# Autodesk Inventor assembly: Chassis-ver1-1111-2021
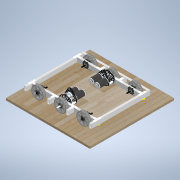
[picture p0: Inventor's stored thumbnail of the model, 180x180]
Saved by Autodesk Inventor 2020 (Build 240168000, 168)
## iProperties
Created: 2021-01-26
Part Number: Chassis-ver1-1111-2021
Document SubType Name: Assembly
Designer: Caitlin
Author: Caitlin
## Documents named in this file (14)
- D:\PHRC CADD 2021\PHRC CADD\2020 Infinite Recharge\2021 Infinite Recharge\Chassis\Chassis-ver1-1111-2021.iam
- D:\PHRC CADD 2021\PHRC CADD\2020 Infinite Recharge\Platform.ver1-1111-2020.ipt
- D:\PHRC CADD 2021\PHRC CADD\2020 Infinite Recharge\Chassis\Parts\2x1 20in Alluminum.ver1-1111-2019.ipt
- D:\PHRC CADD 2021\PHRC CADD\2020 Infinite Recharge\Chassis\Parts\2x1 20in Alluminum with Cal Drop.ver1-1111-2019.ipt
- D:\PHRC CADD 2021\PHRC CADD\Resources\VEXpro Resources\Gussets\ChassisGusset-1111-2016.ipt
- D:\PHRC CADD 2021\PHRC CADD\2020 Infinite Recharge\Chassis\Parts\2x1 2in Alluminum Block.ver1-1111-2019.ipt
- D:\PHRC CADD 2021\PHRC CADD\Resources\VEXpro Resources\Bearings\0.5inHexFlangedBearing(1.125inx0.313in)-1111-2016.ipt
- D:\PHRC CADD 2021\PHRC CADD\Resources\VEXpro Resources\Spacers\0.5inAcetalSpace(0.5inHex)-1111-2016.ipt
- D:\PHRC CADD 2021\PHRC CADD\Resources\VEXpro Resources\Versa Motion\VersaBlockKit-1111-2016.ipt
- D:\PHRC CADD 2021\PHRC CADD\Resources\VEXpro Resources\Gearboxes\WCP SS Gearbox\SS-Gearbox.iam
- D:\PHRC CADD 2021\PHRC CADD\Resources\VEXpro Resources\Shafts\0.5inThunderHexShaft(8)-1111-2016.ipt
- D:\PHRC CADD 2021\PHRC CADD\Resources\VEXpro Resources\Wheels\6 inch\6x1inTractionWheel-1111-2016.iam
- D:\PHRC CADD 2021\PHRC CADD\2020 Infinite Recharge\Chassis\Parts\BumperMount1-ver1-1111-2019.ipt
- D:\PHRC CADD 2021\PHRC CADD\2020 Infinite Recharge\Chassis\Parts\ElectricalBoard.ver2-1111-2020.ipt
## Components (51 placed, 13 different names)
1. Platform.ver1-1111-2020:1 — Mate:1, Flush:1, Flush:2
2. 2x1 20in Alluminum.ver1-1111-2019:1 — Mate:1, Flush:1, Flush:2, Mate:2, Mate:3, Flush:3, Mate:4, Mate:5, Flush:4, Mate:8, Flush:6, Mate:9, Flush:8, Mate:14, Mate:40, Flush:23, Mate:41, Flush:27, Mate:46
3. 2x1 20in Alluminum with Cal Drop.ver1-1111-2019:1 — Mate:2, Mate:3, Flush:3, Mate:6, Mate:7, Flush:5, Flush:7, Flush:11, Mate:12, Mate:13, Mate:15, Mate:16, Flush:14, Mate:19, Flush:16, Cylindrical:3, Mate:30, Cylindrical:4, Mate:31, Cylindrical:7, Mate:34, Cylindrical:8, Mate:35, Angle:5, Angle:6, Angle:7, Angle:8, Cylindrical:9, Mate:36, Angle:13, Flush:25, Flush:26, Mate:43, Mate:44, Mate:45, Flush:28
4. 2x1 20in Alluminum with Cal Drop.ver1-1111-2019:2 — Mate:4, Mate:5, Flush:4, Flush:9, Flush:13, Mate:20, Mate:21, Mate:23, Mate:24, Mate:26, Flush:18, Mate:27, Flush:20, Cylindrical:1, Mate:28, Cylindrical:2, Mate:29, Cylindrical:5, Mate:32, Cylindrical:6, Mate:33, Angle:9, Angle:10, Angle:11, Angle:12, Cylindrical:10, Mate:37, Angle:14, Mate:38, Flush:22, Mate:39, Flush:24, Mate:42
5. 2x1 20in Alluminum.ver1-1111-2019:2 — Mate:6, Mate:7, Flush:5, Mate:10, Flush:10, Mate:11, Flush:12, Mate:22
6. ChassisGusset-1111-2016:1 — Mate:8, Flush:6, Flush:7
7. ChassisGusset-1111-2016:2 — Mate:9, Flush:8, Flush:9
8. ChassisGusset-1111-2016:3 — Mate:10, Flush:10, Flush:11
9. ChassisGusset-1111-2016:4 — Mate:11, Flush:12, Flush:13
10. 2x1 2in Alluminum Block.ver1-1111-2019:1 — Mate:12, Mate:13, Mate:14, Mate:17, Flush:17
11. 2x1 2in Alluminum Block.ver1-1111-2019:2 — Mate:15, Mate:16, Mate:17, Mate:18, Flush:15
12. ChassisGusset-1111-2016:5 — Mate:18, Flush:14, Flush:15
13. ChassisGusset-1111-2016:6 — Mate:19, Flush:16, Flush:17
14. 2x1 2in Alluminum Block.ver1-1111-2019:3 — Mate:20, Mate:21, Mate:22, Mate:25, Flush:19
15. 2x1 2in Alluminum Block.ver1-1111-2019:4 — Mate:23, Mate:24, Mate:25, Flush:21
16. ChassisGusset-1111-2016:7 — Mate:26, Flush:18, Flush:19
17. ChassisGusset-1111-2016:8 — Mate:27, Flush:20, Flush:21
18. 0.5inHexFlangedBearing(1.125inx0.313in)-1111-2016:1 — Cylindrical:1, Mate:28, Rotational:11
19. 0.5inHexFlangedBearing(1.125inx0.313in)-1111-2016:2 — Cylindrical:2, Mate:29, Rotational:12
20. 0.5inHexFlangedBearing(1.125inx0.313in)-1111-2016:3 — Cylindrical:3, Mate:30, Rotational:8
21. 0.5inHexFlangedBearing(1.125inx0.313in)-1111-2016:4 — Cylindrical:4, Mate:31, Rotational:7
22. 0.5inHexFlangedBearing(1.125inx0.313in)-1111-2016:5 — Cylindrical:5, Mate:32, Rotational:3, Angle:3, Rotational:9
23. 0.5inHexFlangedBearing(1.125inx0.313in)-1111-2016:6 — Cylindrical:6, Mate:33, Rotational:4, Angle:4, Rotational:10, Cylindrical:14
24. 0.5inHexFlangedBearing(1.125inx0.313in)-1111-2016:7 — Cylindrical:7, Mate:34, Rotational:1, Angle:1, Rotational:5
25. 0.5inHexFlangedBearing(1.125inx0.313in)-1111-2016:8 — Cylindrical:8, Mate:35, Rotational:2, Angle:2, Rotational:6
26. 0.5inAcetalSpace(0.5inHex)-1111-2016:1 — Rotational:1, Angle:1, Cylindrical:17
27. 0.5inAcetalSpace(0.5inHex)-1111-2016:2 — Rotational:2, Angle:2, Cylindrical:16
28. 0.5inAcetalSpace(0.5inHex)-1111-2016:3 — Rotational:3, Angle:3, Cylindrical:12
29. 0.5inAcetalSpace(0.5inHex)-1111-2016:4 — Rotational:4, Angle:4
30. VersaBlockKit-1111-2016:1 — Rotational:5, Angle:5
31. VersaBlockKit-1111-2016:2 — Rotational:6, Angle:6
32. VersaBlockKit-1111-2016:3 — Rotational:7, Angle:7
33. VersaBlockKit-1111-2016:4 — Rotational:8, Angle:8
34. VersaBlockKit-1111-2016:5 — Rotational:9, Angle:9
35. VersaBlockKit-1111-2016:6 — Rotational:10, Angle:10
36. VersaBlockKit-1111-2016:7 — Rotational:11, Angle:11
37. VersaBlockKit-1111-2016:8 — Rotational:12, Angle:12
38. SS-Gearbox:1 [sub-assembly] — Cylindrical:9, Mate:36, Angle:13, Cylindrical:20
39. SS-Gearbox:2 [sub-assembly] — Cylindrical:10, Mate:37, Angle:14, Cylindrical:11
40. 0.5inThunderHexShaft(8)-1111-2016:1 — Cylindrical:12, Flush:22, Cylindrical:13, Angle:15
41. 6x1inTractionWheel-1111-2016:1 [sub-assembly] — Cylindrical:11, Mate:38
42. 6x1inTractionWheel-1111-2016:2 [sub-assembly] — Cylindrical:13, Mate:39, Angle:15
43. BumperMount1-ver1-1111-2019:1 — Mate:40, Flush:23, Mate:41
44. 0.5inThunderHexShaft(8)-1111-2016:2 — Cylindrical:14, Flush:24, Cylindrical:15, Angle:16
45. 6x1inTractionWheel-1111-2016:3 [sub-assembly] — Cylindrical:15, Mate:42, Angle:16
46. 0.5inThunderHexShaft(8)-1111-2016:3 — Cylindrical:16, Flush:25, Cylindrical:18, Angle:17
47. 0.5inThunderHexShaft(8)-1111-2016:4 — Cylindrical:17, Flush:26, Cylindrical:19, Angle:18
48. 6x1inTractionWheel-1111-2016:4 [sub-assembly] — Cylindrical:18, Mate:43, Angle:17
49. 6x1inTractionWheel-1111-2016:5 [sub-assembly] — Cylindrical:19, Mate:44, Angle:18
50. 6x1inTractionWheel-1111-2016:6 [sub-assembly] — Cylindrical:20, Mate:45
51. ElectricalBoard.ver2-1111-2020:1 — Flush:27, Mate:46, Flush:28
## Relationships (124: Mate 46, Flush 28, CylindricalJoint 20, Angle 18, RevoluteJoint 12)
- Mate:1 (47.625 mm): Platform.ver1-1111-2020:1 ↔ 2x1 20in Alluminum.ver1-1111-2019:1
- Flush:1 (141.605 mm): Platform.ver1-1111-2020:1 ↔ 2x1 20in Alluminum.ver1-1111-2019:1
- Flush:2 (127 mm): Platform.ver1-1111-2020:1 ↔ 2x1 20in Alluminum.ver1-1111-2019:1
- Mate:2: 2x1 20in Alluminum.ver1-1111-2019:1 ↔ 2x1 20in Alluminum with Cal Drop.ver1-1111-2019:1
- Mate:3: 2x1 20in Alluminum.ver1-1111-2019:1 ↔ 2x1 20in Alluminum with Cal Drop.ver1-1111-2019:1
- Flush:3 (69.85 mm): 2x1 20in Alluminum.ver1-1111-2019:1 ↔ 2x1 20in Alluminum with Cal Drop.ver1-1111-2019:1
- Mate:4: 2x1 20in Alluminum.ver1-1111-2019:1 ↔ 2x1 20in Alluminum with Cal Drop.ver1-1111-2019:2
- Mate:5: 2x1 20in Alluminum.ver1-1111-2019:1 ↔ 2x1 20in Alluminum with Cal Drop.ver1-1111-2019:2
- Flush:4 (69.85 mm): 2x1 20in Alluminum.ver1-1111-2019:1 ↔ 2x1 20in Alluminum with Cal Drop.ver1-1111-2019:2
- Mate:6: 2x1 20in Alluminum with Cal Drop.ver1-1111-2019:1 ↔ 2x1 20in Alluminum.ver1-1111-2019:2
- Mate:7: 2x1 20in Alluminum with Cal Drop.ver1-1111-2019:1 ↔ 2x1 20in Alluminum.ver1-1111-2019:2
- Flush:5 (69.85 mm): 2x1 20in Alluminum with Cal Drop.ver1-1111-2019:1 ↔ 2x1 20in Alluminum.ver1-1111-2019:2
- Mate:8: 2x1 20in Alluminum.ver1-1111-2019:1 ↔ ChassisGusset-1111-2016:1
- Flush:6: 2x1 20in Alluminum.ver1-1111-2019:1 ↔ ChassisGusset-1111-2016:1
- Flush:7: 2x1 20in Alluminum with Cal Drop.ver1-1111-2019:1 ↔ ChassisGusset-1111-2016:1
- Mate:9: 2x1 20in Alluminum.ver1-1111-2019:1 ↔ ChassisGusset-1111-2016:2
- Flush:8: 2x1 20in Alluminum.ver1-1111-2019:1 ↔ ChassisGusset-1111-2016:2
- Flush:9: 2x1 20in Alluminum with Cal Drop.ver1-1111-2019:2 ↔ ChassisGusset-1111-2016:2
- Mate:10: 2x1 20in Alluminum.ver1-1111-2019:2 ↔ ChassisGusset-1111-2016:3
- Flush:10: 2x1 20in Alluminum.ver1-1111-2019:2 ↔ ChassisGusset-1111-2016:3
- Flush:11: 2x1 20in Alluminum with Cal Drop.ver1-1111-2019:1 ↔ ChassisGusset-1111-2016:3
- Mate:11: 2x1 20in Alluminum.ver1-1111-2019:2 ↔ ChassisGusset-1111-2016:4
- Flush:12: 2x1 20in Alluminum.ver1-1111-2019:2 ↔ ChassisGusset-1111-2016:4
- Flush:13: 2x1 20in Alluminum with Cal Drop.ver1-1111-2019:2 ↔ ChassisGusset-1111-2016:4
- Mate:12: 2x1 20in Alluminum with Cal Drop.ver1-1111-2019:1 ↔ 2x1 2in Alluminum Block.ver1-1111-2019:1
- Mate:13: 2x1 20in Alluminum with Cal Drop.ver1-1111-2019:1 ↔ 2x1 2in Alluminum Block.ver1-1111-2019:1
- Mate:14 (254 mm): 2x1 20in Alluminum.ver1-1111-2019:1 ↔ 2x1 2in Alluminum Block.ver1-1111-2019:1
- Mate:15: 2x1 20in Alluminum with Cal Drop.ver1-1111-2019:1 ↔ 2x1 2in Alluminum Block.ver1-1111-2019:2
- Mate:16: 2x1 20in Alluminum with Cal Drop.ver1-1111-2019:1 ↔ 2x1 2in Alluminum Block.ver1-1111-2019:2
- Mate:17 (203.2 mm): 2x1 2in Alluminum Block.ver1-1111-2019:1 ↔ 2x1 2in Alluminum Block.ver1-1111-2019:2
- Mate:18: 2x1 2in Alluminum Block.ver1-1111-2019:2 ↔ ChassisGusset-1111-2016:5
- Flush:14: 2x1 20in Alluminum with Cal Drop.ver1-1111-2019:1 ↔ ChassisGusset-1111-2016:5
- Flush:15: 2x1 2in Alluminum Block.ver1-1111-2019:2 ↔ ChassisGusset-1111-2016:5
- Mate:19: 2x1 20in Alluminum with Cal Drop.ver1-1111-2019:1 ↔ ChassisGusset-1111-2016:6
- Flush:16: 2x1 20in Alluminum with Cal Drop.ver1-1111-2019:1 ↔ ChassisGusset-1111-2016:6
- Flush:17: 2x1 2in Alluminum Block.ver1-1111-2019:1 ↔ ChassisGusset-1111-2016:6
- Mate:20: 2x1 20in Alluminum with Cal Drop.ver1-1111-2019:2 ↔ 2x1 2in Alluminum Block.ver1-1111-2019:3
- Mate:21: 2x1 20in Alluminum with Cal Drop.ver1-1111-2019:2 ↔ 2x1 2in Alluminum Block.ver1-1111-2019:3
- Mate:22 (254 mm): 2x1 20in Alluminum.ver1-1111-2019:2 ↔ 2x1 2in Alluminum Block.ver1-1111-2019:3
- Mate:23: 2x1 20in Alluminum with Cal Drop.ver1-1111-2019:2 ↔ 2x1 2in Alluminum Block.ver1-1111-2019:4
- Mate:24: 2x1 20in Alluminum with Cal Drop.ver1-1111-2019:2 ↔ 2x1 2in Alluminum Block.ver1-1111-2019:4
- Mate:25 (203.2 mm): 2x1 2in Alluminum Block.ver1-1111-2019:3 ↔ 2x1 2in Alluminum Block.ver1-1111-2019:4
- Mate:26: 2x1 20in Alluminum with Cal Drop.ver1-1111-2019:2 ↔ ChassisGusset-1111-2016:7
- Flush:18: 2x1 20in Alluminum with Cal Drop.ver1-1111-2019:2 ↔ ChassisGusset-1111-2016:7
- Flush:19: 2x1 2in Alluminum Block.ver1-1111-2019:3 ↔ ChassisGusset-1111-2016:7
- Mate:27: 2x1 20in Alluminum with Cal Drop.ver1-1111-2019:2 ↔ ChassisGusset-1111-2016:8
- Flush:20: 2x1 20in Alluminum with Cal Drop.ver1-1111-2019:2 ↔ ChassisGusset-1111-2016:8
- Flush:21: 2x1 2in Alluminum Block.ver1-1111-2019:4 ↔ ChassisGusset-1111-2016:8
- Cylindrical:1: 2x1 20in Alluminum with Cal Drop.ver1-1111-2019:2 ↔ 0.5inHexFlangedBearing(1.125inx0.313in)-1111-2016:1
- Mate:28 (6.35 mm): 2x1 20in Alluminum with Cal Drop.ver1-1111-2019:2 ↔ 0.5inHexFlangedBearing(1.125inx0.313in)-1111-2016:1
- Cylindrical:2: 2x1 20in Alluminum with Cal Drop.ver1-1111-2019:2 ↔ 0.5inHexFlangedBearing(1.125inx0.313in)-1111-2016:2
- Mate:29 (6.35 mm): 2x1 20in Alluminum with Cal Drop.ver1-1111-2019:2 ↔ 0.5inHexFlangedBearing(1.125inx0.313in)-1111-2016:2
- Cylindrical:3: 2x1 20in Alluminum with Cal Drop.ver1-1111-2019:1 ↔ 0.5inHexFlangedBearing(1.125inx0.313in)-1111-2016:3
- Mate:30 (6.35 mm): 2x1 20in Alluminum with Cal Drop.ver1-1111-2019:1 ↔ 0.5inHexFlangedBearing(1.125inx0.313in)-1111-2016:3
- Cylindrical:4: 2x1 20in Alluminum with Cal Drop.ver1-1111-2019:1 ↔ 0.5inHexFlangedBearing(1.125inx0.313in)-1111-2016:4
- Mate:31 (6.35 mm): 2x1 20in Alluminum with Cal Drop.ver1-1111-2019:1 ↔ 0.5inHexFlangedBearing(1.125inx0.313in)-1111-2016:4
- Cylindrical:5: 2x1 20in Alluminum with Cal Drop.ver1-1111-2019:2 ↔ 0.5inHexFlangedBearing(1.125inx0.313in)-1111-2016:5
- Mate:32 (6.35 mm): 2x1 20in Alluminum with Cal Drop.ver1-1111-2019:2 ↔ 0.5inHexFlangedBearing(1.125inx0.313in)-1111-2016:5
- Cylindrical:6: 2x1 20in Alluminum with Cal Drop.ver1-1111-2019:2 ↔ 0.5inHexFlangedBearing(1.125inx0.313in)-1111-2016:6
- Mate:33 (6.35 mm): 2x1 20in Alluminum with Cal Drop.ver1-1111-2019:2 ↔ 0.5inHexFlangedBearing(1.125inx0.313in)-1111-2016:6
- Cylindrical:7: 2x1 20in Alluminum with Cal Drop.ver1-1111-2019:1 ↔ 0.5inHexFlangedBearing(1.125inx0.313in)-1111-2016:7
- Mate:34 (6.35 mm): 2x1 20in Alluminum with Cal Drop.ver1-1111-2019:1 ↔ 0.5inHexFlangedBearing(1.125inx0.313in)-1111-2016:7
- Cylindrical:8: 2x1 20in Alluminum with Cal Drop.ver1-1111-2019:1 ↔ 0.5inHexFlangedBearing(1.125inx0.313in)-1111-2016:8
- Mate:35 (6.35 mm): 2x1 20in Alluminum with Cal Drop.ver1-1111-2019:1 ↔ 0.5inHexFlangedBearing(1.125inx0.313in)-1111-2016:8
- Rotational:1 [RevoluteJoint] (5.969 mm): 0.5inHexFlangedBearing(1.125inx0.313in)-1111-2016:7 ↔ 0.5inAcetalSpace(0.5inHex)-1111-2016:1
- Angle:1 (0 deg): 0.5inHexFlangedBearing(1.125inx0.313in)-1111-2016:7 ↔ 0.5inAcetalSpace(0.5inHex)-1111-2016:1
- Rotational:2 [RevoluteJoint] (5.969 mm): 0.5inHexFlangedBearing(1.125inx0.313in)-1111-2016:8 ↔ 0.5inAcetalSpace(0.5inHex)-1111-2016:2
- Angle:2 (0 deg): 0.5inHexFlangedBearing(1.125inx0.313in)-1111-2016:8 ↔ 0.5inAcetalSpace(0.5inHex)-1111-2016:2
- Rotational:3 [RevoluteJoint] (5.969 mm): 0.5inHexFlangedBearing(1.125inx0.313in)-1111-2016:5 ↔ 0.5inAcetalSpace(0.5inHex)-1111-2016:3
- Angle:3 (0 deg): 0.5inHexFlangedBearing(1.125inx0.313in)-1111-2016:5 ↔ 0.5inAcetalSpace(0.5inHex)-1111-2016:3
- Rotational:4 [RevoluteJoint] (5.969 mm): 0.5inHexFlangedBearing(1.125inx0.313in)-1111-2016:6 ↔ 0.5inAcetalSpace(0.5inHex)-1111-2016:4
- Angle:4 (0 deg): 0.5inHexFlangedBearing(1.125inx0.313in)-1111-2016:6 ↔ 0.5inAcetalSpace(0.5inHex)-1111-2016:4
- Rotational:5 [RevoluteJoint]: 0.5inHexFlangedBearing(1.125inx0.313in)-1111-2016:7 ↔ VersaBlockKit-1111-2016:1
- Angle:5 (0 deg): 2x1 20in Alluminum with Cal Drop.ver1-1111-2019:1 ↔ VersaBlockKit-1111-2016:1
- Rotational:6 [RevoluteJoint]: 0.5inHexFlangedBearing(1.125inx0.313in)-1111-2016:8 ↔ VersaBlockKit-1111-2016:2
- Angle:6 (0 deg): 2x1 20in Alluminum with Cal Drop.ver1-1111-2019:1 ↔ VersaBlockKit-1111-2016:2
- Rotational:7 [RevoluteJoint]: 0.5inHexFlangedBearing(1.125inx0.313in)-1111-2016:4 ↔ VersaBlockKit-1111-2016:3
- Angle:7 (0 deg): 2x1 20in Alluminum with Cal Drop.ver1-1111-2019:1 ↔ VersaBlockKit-1111-2016:3
- Rotational:8 [RevoluteJoint]: 0.5inHexFlangedBearing(1.125inx0.313in)-1111-2016:3 ↔ VersaBlockKit-1111-2016:4
- Angle:8 (0 deg): 2x1 20in Alluminum with Cal Drop.ver1-1111-2019:1 ↔ VersaBlockKit-1111-2016:4
- Rotational:9 [RevoluteJoint]: 0.5inHexFlangedBearing(1.125inx0.313in)-1111-2016:5 ↔ VersaBlockKit-1111-2016:5
- Angle:9 (0 deg): 2x1 20in Alluminum with Cal Drop.ver1-1111-2019:2 ↔ VersaBlockKit-1111-2016:5
- Rotational:10 [RevoluteJoint]: 0.5inHexFlangedBearing(1.125inx0.313in)-1111-2016:6 ↔ VersaBlockKit-1111-2016:6
- Angle:10 (0 deg): 2x1 20in Alluminum with Cal Drop.ver1-1111-2019:2 ↔ VersaBlockKit-1111-2016:6
- Rotational:11 [RevoluteJoint]: 0.5inHexFlangedBearing(1.125inx0.313in)-1111-2016:1 ↔ VersaBlockKit-1111-2016:7
- Angle:11 (0 deg): 2x1 20in Alluminum with Cal Drop.ver1-1111-2019:2 ↔ VersaBlockKit-1111-2016:7
- Rotational:12 [RevoluteJoint]: 0.5inHexFlangedBearing(1.125inx0.313in)-1111-2016:2 ↔ VersaBlockKit-1111-2016:8
- Angle:12 (0 deg): 2x1 20in Alluminum with Cal Drop.ver1-1111-2019:2 ↔ VersaBlockKit-1111-2016:8
- Cylindrical:9: 2x1 20in Alluminum with Cal Drop.ver1-1111-2019:1 ↔ SS-Gearbox:1
- Mate:36: 2x1 20in Alluminum with Cal Drop.ver1-1111-2019:1 ↔ SS-Gearbox:1
- Angle:13 (0 deg): 2x1 20in Alluminum with Cal Drop.ver1-1111-2019:1 ↔ SS-Gearbox:1
- Cylindrical:10: 2x1 20in Alluminum with Cal Drop.ver1-1111-2019:2 ↔ SS-Gearbox:2
- Mate:37: 2x1 20in Alluminum with Cal Drop.ver1-1111-2019:2 ↔ SS-Gearbox:2
- Angle:14 (0 deg): 2x1 20in Alluminum with Cal Drop.ver1-1111-2019:2 ↔ SS-Gearbox:2
- Cylindrical:11: SS-Gearbox:2 ↔ 6x1inTractionWheel-1111-2016:1
- Mate:38 (7.9502 mm): 2x1 20in Alluminum with Cal Drop.ver1-1111-2019:2 ↔ 6x1inTractionWheel-1111-2016:1
- Cylindrical:12: 0.5inAcetalSpace(0.5inHex)-1111-2016:3 ↔ 0.5inThunderHexShaft(8)-1111-2016:1
- Flush:22 (-52.4002 mm): 2x1 20in Alluminum with Cal Drop.ver1-1111-2019:2 ↔ 0.5inThunderHexShaft(8)-1111-2016:1
- Cylindrical:13: 0.5inThunderHexShaft(8)-1111-2016:1 ↔ 6x1inTractionWheel-1111-2016:2
- Mate:39 (9.9822 mm): 2x1 20in Alluminum with Cal Drop.ver1-1111-2019:2 ↔ 6x1inTractionWheel-1111-2016:2
- Angle:15 (0 deg): 0.5inThunderHexShaft(8)-1111-2016:1 ↔ 6x1inTractionWheel-1111-2016:2
- Mate:40: 2x1 20in Alluminum.ver1-1111-2019:1 ↔ BumperMount1-ver1-1111-2019:1
- Flush:23: 2x1 20in Alluminum.ver1-1111-2019:1 ↔ BumperMount1-ver1-1111-2019:1
- Mate:41: 2x1 20in Alluminum.ver1-1111-2019:1 ↔ BumperMount1-ver1-1111-2019:1
- Cylindrical:14: 0.5inHexFlangedBearing(1.125inx0.313in)-1111-2016:6 ↔ 0.5inThunderHexShaft(8)-1111-2016:2
- Flush:24 (-51.7144 mm): 2x1 20in Alluminum with Cal Drop.ver1-1111-2019:2 ↔ 0.5inThunderHexShaft(8)-1111-2016:2
- Cylindrical:15: 0.5inThunderHexShaft(8)-1111-2016:2 ↔ 6x1inTractionWheel-1111-2016:3
- Mate:42 (9.9822 mm): 2x1 20in Alluminum with Cal Drop.ver1-1111-2019:2 ↔ 6x1inTractionWheel-1111-2016:3
- Angle:16 (0 deg): 0.5inThunderHexShaft(8)-1111-2016:2 ↔ 6x1inTractionWheel-1111-2016:3
- Cylindrical:16: 0.5inAcetalSpace(0.5inHex)-1111-2016:2 ↔ 0.5inThunderHexShaft(8)-1111-2016:3
- Flush:25 (-52.4002 mm): 2x1 20in Alluminum with Cal Drop.ver1-1111-2019:1 ↔ 0.5inThunderHexShaft(8)-1111-2016:3
- Cylindrical:17: 0.5inAcetalSpace(0.5inHex)-1111-2016:1 ↔ 0.5inThunderHexShaft(8)-1111-2016:4
- Flush:26 (-52.4002 mm): 2x1 20in Alluminum with Cal Drop.ver1-1111-2019:1 ↔ 0.5inThunderHexShaft(8)-1111-2016:4
- Cylindrical:18: 0.5inThunderHexShaft(8)-1111-2016:3 ↔ 6x1inTractionWheel-1111-2016:4
- Mate:43 (9.9822 mm): 2x1 20in Alluminum with Cal Drop.ver1-1111-2019:1 ↔ 6x1inTractionWheel-1111-2016:4
- Angle:17 (0 deg): 0.5inThunderHexShaft(8)-1111-2016:3 ↔ 6x1inTractionWheel-1111-2016:4
- Cylindrical:19: 0.5inThunderHexShaft(8)-1111-2016:4 ↔ 6x1inTractionWheel-1111-2016:5
- Mate:44 (9.9822 mm): 2x1 20in Alluminum with Cal Drop.ver1-1111-2019:1 ↔ 6x1inTractionWheel-1111-2016:5
- Angle:18 (0 deg): 0.5inThunderHexShaft(8)-1111-2016:4 ↔ 6x1inTractionWheel-1111-2016:5
- Cylindrical:20: SS-Gearbox:1 ↔ 6x1inTractionWheel-1111-2016:6
- Mate:45 (7.9502 mm): 2x1 20in Alluminum with Cal Drop.ver1-1111-2019:1 ↔ 6x1inTractionWheel-1111-2016:6
- Flush:27: 2x1 20in Alluminum.ver1-1111-2019:1 ↔ ElectricalBoard.ver2-1111-2020:1
- Mate:46: 2x1 20in Alluminum.ver1-1111-2019:1 ↔ ElectricalBoard.ver2-1111-2020:1
- Flush:28 (-12.7 mm): 2x1 20in Alluminum with Cal Drop.ver1-1111-2019:1 ↔ ElectricalBoard.ver2-1111-2020:1
